# Autodesk Inventor assembly: 40-J4
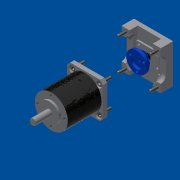
[picture p0: Inventor's stored thumbnail of the model, 180x180]
Saved by Autodesk Inventor 2018 (Build 220112000, 112)
## iProperties
Created: 2020-06-07
Part Number: 40-J4
Document SubType Name: Assembly
Designer: Bunny320
Author: Bunny320
## Documents named in this file (2)
- C:\Users\Bunny320\Desktop\sechs\4-CAD\40-J4.iam
- C:\Users\Bunny320\Desktop\sechs\4-CAD\motor unit 2820.iam
## Components (1 placed, 1 different names)
1. motor unit 2820:1 [sub-assembly] — Flush:1, Flush:2, Flush:3
## Relationships (3: Flush 3)
- Flush:1: motor unit 2820:1
- Flush:2: motor unit 2820:1
- Flush:3: motor unit 2820:1
